# Autodesk Inventor assembly: Assembly3
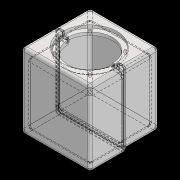
[picture p0: Inventor's stored thumbnail of the model, 180x180]
Saved by Autodesk Inventor 2022 (Build 260153000, 153)
## iProperties
Created: 2022-07-08
Part Number: Assembly3
Document SubType Name: Assembly
Designer: Fuzzyfish
Author: Fuzzyfish
## Documents named in this file (3)
- C:\Users\Fuzzyfish\Documents\Inventor\finalBox\Assembly3.iam
- C:\Users\Fuzzyfish\Documents\Inventor\finalBox\chonkyWoofer\groove.ipt
- C:\Users\Fuzzyfish\Documents\Inventor\finalBox\chonkyWoofer\tonguev2.ipt
## Components (2 placed, 2 different names)
1. groove:1 — Flush:1, Flush:2, Mate:1
2. tonguev2:1 — Flush:1, Flush:2, Mate:1
## Relationships (3: Flush 2, Mate 1)
- Flush:1: groove:1 ↔ tonguev2:1
- Flush:2: groove:1 ↔ tonguev2:1
- Mate:1: groove:1 ↔ tonguev2:1
